# Autodesk Inventor assembly: 2924-1015-1000 assembly
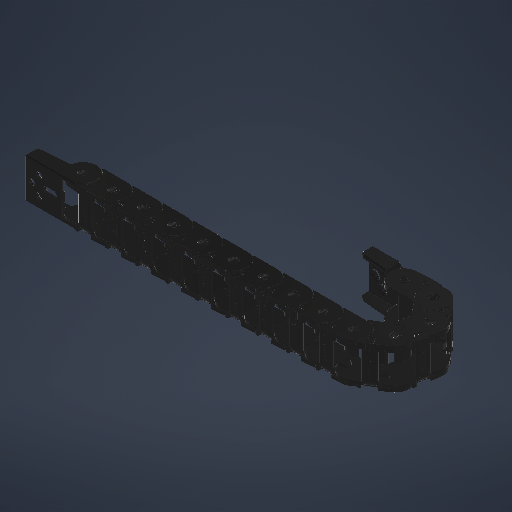
[picture p0: Inventor's stored thumbnail of the model, 512x512]
Saved by Autodesk Inventor 2026.2 (Build 302298000, 298)
## iProperties
Created: 2023-10-18
Part Number: 2924-1015-1000 assembly
Description: STEP AP203
Document SubType Name: Assembly
Designer: Kenji
Sending System: SolidWorks 2016
Preprocessor: SwSTEP 2.0
Title: 2924-1015-1000 assembly.STEP
Revision Number: ANY
## Documents named in this file (4)
- C:\Users\Kenji\Documents\GitHub\DiyCNC-\COTS-Parts\10x15-CableCarrierZAxis-2924-1015-1000.iam
- C:\Users\Kenji\Downloads\2924-1015-1000\2924-1015-1000 assembly\2924-1015-1000 assembly\2924-1015 End 1.ipt
- C:\Users\Kenji\Downloads\2924-1015-1000\2924-1015-1000 assembly\2924-1015-1000 assembly\2924-1015 link.ipt
- C:\Users\Kenji\Downloads\2924-1015-1000\2924-1015-1000 assembly\2924-1015-1000 assembly\2924-1015 End 2.ipt
## Components (15 placed, 12 different names)
1. 2924-1015 End 1_1 — Mate:1, Mate:5, Mate:6, Angle:1
2. 2924-1015 link_2 — Mate:1, Mate:4, Mate:5, Mate:6, Mate:7, Mate:8
3. 2924-1015 link_3 — Mate:12, Mate:13, Mate:14, Mate:15, Mate:16
4. 2924-1015 link_4 — Mate:4, Mate:7, Mate:8, Mate:9, Mate:10, Mate:11
5. 2924-1015 link_5 — Mate:9, Mate:10, Mate:11, Mate:12, Mate:13, Mate:14
6. 2924-1015 link_6 — Mate:15, Mate:16, Angle:1, Mate:17, Mate:18, Flush:1
7. 2924-1015 link_7 — Mate:17, Mate:18, Flush:1, Mate:19, Mate:20, Flush:2
8. 2924-1015 link_8 — Mate:19, Mate:20, Flush:2, Mate:21, Mate:22, Flush:3
9. 2924-1015 link_9 — Mate:21, Mate:22, Flush:3, Mate:23, Mate:24, Flush:4
10. 2924-1015 End 2_59 — Mate:25, Mate:26, Angle:2
11. 2924-1015 link_10 — Mate:23, Mate:24, Flush:4
12. 2924-1015 link:58
13. 2924-1015 link:59
14. 2924-1015 link:60
15. 2924-1015 link:61 — Mate:25, Mate:26, Angle:2
## Component patterns: (5 elements, first: 2924-1015 link_10)
## Relationships (30: Mate 24, Flush 4, Angle 2)
- Mate:1: 2924-1015 End 1_1 ↔ 2924-1015 link_2
- Mate:4: 2924-1015 link_2 ↔ 2924-1015 link_4
- Mate:5: 2924-1015 End 1_1 ↔ 2924-1015 link_2
- Mate:6: 2924-1015 End 1_1 ↔ 2924-1015 link_2
- Mate:7: 2924-1015 link_2 ↔ 2924-1015 link_4
- Mate:8: 2924-1015 link_2 ↔ 2924-1015 link_4
- Mate:9: 2924-1015 link_4 ↔ 2924-1015 link_5
- Mate:10: 2924-1015 link_4 ↔ 2924-1015 link_5
- Mate:11: 2924-1015 link_4 ↔ 2924-1015 link_5
- Mate:12: 2924-1015 link_3 ↔ 2924-1015 link_5
- Mate:13: 2924-1015 link_3 ↔ 2924-1015 link_5
- Mate:14: 2924-1015 link_3 ↔ 2924-1015 link_5
- Mate:15: 2924-1015 link_3 ↔ 2924-1015 link_6
- Mate:16: 2924-1015 link_3 ↔ 2924-1015 link_6
- Angle:1 (0 deg): 2924-1015 End 1_1 ↔ 2924-1015 link_6
- Mate:17: 2924-1015 link_6 ↔ 2924-1015 link_7
- Mate:18: 2924-1015 link_6 ↔ 2924-1015 link_7
- Flush:1: 2924-1015 link_6 ↔ 2924-1015 link_7
- Mate:19: 2924-1015 link_7 ↔ 2924-1015 link_8
- Mate:20: 2924-1015 link_7 ↔ 2924-1015 link_8
- Flush:2: 2924-1015 link_7 ↔ 2924-1015 link_8
- Mate:21: 2924-1015 link_8 ↔ 2924-1015 link_9
- Mate:22: 2924-1015 link_8 ↔ 2924-1015 link_9
- Flush:3: 2924-1015 link_8 ↔ 2924-1015 link_9
- Mate:23: 2924-1015 link_9 ↔ 2924-1015 link_10
- Mate:24: 2924-1015 link_9 ↔ 2924-1015 link_10
- Flush:4: 2924-1015 link_9 ↔ 2924-1015 link_10
- Mate:25: 2924-1015 End 2_59 ↔ 2924-1015 link:61
- Mate:26: 2924-1015 End 2_59 ↔ 2924-1015 link:61
- Angle:2 (0 deg): 2924-1015 End 2_59 ↔ 2924-1015 link:61
